# Autodesk Inventor assembly: Servo Assembly
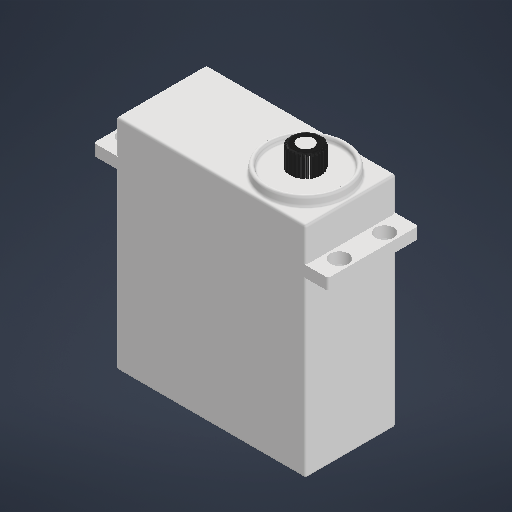
[picture p0: Inventor's stored thumbnail of the model, 512x512]
Saved by Autodesk Inventor 2026.2 (Build 302298010, 298A)
## iProperties
Created: 2026-07-22
Part Number: Servo Assembly
Document SubType Name: Assembly
Designer: Entity
Author: Entity
## Documents named in this file (3)
- C:\Users\Entity\OneDrive\Documents\Bells University of Technology Documents\Autodesk Inventor Projects\Servo Assembly.iam
- C:\Users\Entity\OneDrive\Documents\Bells University of Technology Documents\Autodesk Inventor Projects\Servo Part 1.ipt
- C:\Users\Entity\OneDrive\Documents\Bells University of Technology Documents\Autodesk Inventor Projects\Servo Part 2.ipt
## Components (2 placed, 2 different names)
1. Servo Part 1:1 — Rotational:1
2. Servo Part 2:1 — Rotational:1
## Relationships (1: RevoluteJoint 1)
- Rotational:1 [RevoluteJoint]: Servo Part 1:1 ↔ Servo Part 2:1
